# Autodesk Inventor assembly: GE-17101_ASM_13_ASM
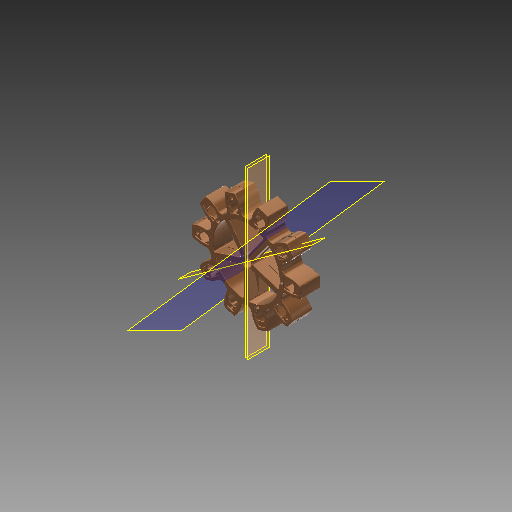
[picture p0: Inventor's stored thumbnail of the model, 512x512]
Saved by Autodesk Inventor 2017 SP1 (Build 210196100, 196)
## iProperties
Created: 2016-12-16
Part Number: GE-17101_ASM_13_ASM
Document SubType Name: Assembly
Designer: PhillipD
Author: PhillipD
Revision Number: 1LAST_VERSION
## Documents named in this file (2)
- D:\snobotics\autodesk\2017\FRC_2017_Field\Parts\GE-17101_ASM_13_ASM.iam
- D:\snobotics\autodesk\2017\FRC_2017_Field\Parts\GE-17100_2.ipt
## Components (2 placed, 2 different names)
1. GE-17100_2_1311 — Mate:4, Mate:5, Mate:6, Mate:7, Mate:8
2. GE-17100_2_1312 — Mate:9
## Relationships (7: Mate 6, Flush 1)
- Mate:4: GE-17100_2_1311
- Mate:5: GE-17100_2_1311
- Mate:6: GE-17100_2_1311
- Mate:7: GE-17100_2_1311
- Mate:8: GE-17100_2_1311
- Mate:9: GE-17100_2_1312
- Flush:1 (6.985 mm)
